# Autodesk Inventor assembly: CardGuideArray
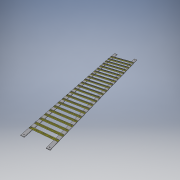
[picture p0: Inventor's stored thumbnail of the model, 180x180]
Saved by Autodesk Inventor 2018 (Build 220112000, 112)
## iProperties
Created: 2025-02-19
Part Number: CardGuideArray
Material: Všeobecné
Document SubType Name: Assembly
Designer: Jozko Mrkvicka
Author: Jozko Mrkvicka
## Documents named in this file (5)
- D:\05_Projekty\Projects_Inventor\Haluska9000\CardGuideArray-4-Inch.iam
- D:\05_Projekty\Projects_Inventor\Haluska9000\CardGuide.ipt
- D:\05_Projekty\Projects_Inventor\Haluska9000\Profile-Flat.ipt
- D:\05_Projekty\Projects_Inventor\Haluska9000\Profile-Flat\Profile-Flat#Cabinet-FerriteCore-Width.ipt
- D:\05_Projekty\Projects_Inventor\Haluska9000\CardGuide\CardGuide#4-inch.ipt
## Components (25 placed, 2 different names)
1. CardGuide#4-inch:1 — Proti sobě:3, Proti sobě:5, Proti sobě:91
2. Profile-Flat#Cabinet-FerriteCore-Width — Stejný směr:1, Stejný směr:2, Proti sobě:3, Proti sobě:5, Proti sobě:6, Proti sobě:7, Proti sobě:8, Proti sobě:9, Proti sobě:10, Proti sobě:11, Proti sobě:12, Proti sobě:13, Proti sobě:14, Proti sobě:15, Proti sobě:16, Proti sobě:17, Proti sobě:19, Proti sobě:20, Proti sobě:22, Proti sobě:23, Proti sobě:24, Proti sobě:25, Proti sobě:26, Proti sobě:27, Proti sobě:28, Proti sobě:29, Proti sobě:52, Proti sobě:53, Proti sobě:55, Proti sobě:56, Proti sobě:57, Proti sobě:58, Proti sobě:60, Proti sobě:73, Proti sobě:89, Proti sobě:94, Proti sobě:97, Proti sobě:101, Proti sobě:102
3. Profile-Flat#Cabinet-FerriteCore-Width:2 — Stejný směr:1, Stejný směr:2, Proti sobě:42, Proti sobě:43, Proti sobě:44, Proti sobě:45, Proti sobě:46, Proti sobě:47, Proti sobě:48, Proti sobě:50, Proti sobě:51, Proti sobě:72, Proti sobě:74, Proti sobě:77, Proti sobě:78, Proti sobě:79, Proti sobě:80, Proti sobě:81, Proti sobě:82, Proti sobě:83, Proti sobě:84, Proti sobě:85, Proti sobě:86, Proti sobě:87, Proti sobě:88, Proti sobě:90, Proti sobě:91, Proti sobě:92, Proti sobě:93, Proti sobě:95, Proti sobě:96, Proti sobě:98, Proti sobě:99, Proti sobě:100
4. CardGuide#4-inch:2 — Proti sobě:6, Proti sobě:19, Proti sobě:92
5. CardGuide#4-inch:3 — Proti sobě:7, Proti sobě:20, Proti sobě:87
6. CardGuide#4-inch:4 — Proti sobě:8, Proti sobě:29, Proti sobě:79
7. CardGuide#4-inch:5 — Proti sobě:9, Proti sobě:93, Proti sobě:94
8. CardGuide#4-inch:6 — Proti sobě:10, Proti sobě:88, Proti sobě:89
9. CardGuide#4-inch:7 — Proti sobě:11, Proti sobě:28, Proti sobě:80
10. CardGuide#4-inch:8 — Proti sobě:12, Proti sobě:27, Proti sobě:81
11. CardGuide#4-inch:9 — Proti sobě:13, Proti sobě:22, Proti sobě:86
12. CardGuide#4-inch:10 — Proti sobě:14, Proti sobě:26, Proti sobě:82
13. CardGuide#4-inch:11 — Proti sobě:15, Proti sobě:23, Proti sobě:83
14. CardGuide#4-inch:12 — Proti sobě:16, Proti sobě:25, Proti sobě:85
15. CardGuide#4-inch:13 — Proti sobě:17, Proti sobě:24, Proti sobě:84
16. CardGuide#4-inch:14 — Proti sobě:42, Proti sobě:52, Proti sobě:99
17. CardGuide#4-inch:15 — Proti sobě:44, Proti sobě:96, Proti sobě:97
18. CardGuide#4-inch:16 — Proti sobě:45, Proti sobě:55, Proti sobě:95
19. CardGuide#4-inch:17 — Proti sobě:43, Proti sobě:53, Proti sobě:98
20. CardGuide#4-inch:18 — Proti sobě:46, Proti sobě:56, Proti sobě:90
21. CardGuide#4-inch:19 — Proti sobě:48, Proti sobě:57, Proti sobě:78
22. CardGuide#4-inch:21 — Proti sobě:50, Proti sobě:60, Proti sobě:74
23. CardGuide#4-inch:22 — Proti sobě:47, Proti sobě:58, Proti sobě:77
24. CardGuide#4-inch:23 — Proti sobě:51, Proti sobě:72, Proti sobě:73
25. CardGuide#4-inch:24 — Proti sobě:100, Proti sobě:101, Proti sobě:102
## Relationships (71: Mate 69, Flush 2)
- Stejný směr:1 [Flush]: Profile-Flat#Cabinet-FerriteCore-Width ↔ Profile-Flat#Cabinet-FerriteCore-Width:2
- Stejný směr:2 [Flush]: Profile-Flat#Cabinet-FerriteCore-Width ↔ Profile-Flat#Cabinet-FerriteCore-Width:2
- Proti sobě:3 [Mate]: CardGuide#4-inch:1 ↔ Profile-Flat#Cabinet-FerriteCore-Width
- Proti sobě:5 [Mate]: CardGuide#4-inch:1 ↔ Profile-Flat#Cabinet-FerriteCore-Width
- Proti sobě:6 [Mate]: Profile-Flat#Cabinet-FerriteCore-Width ↔ CardGuide#4-inch:2
- Proti sobě:7 [Mate]: Profile-Flat#Cabinet-FerriteCore-Width ↔ CardGuide#4-inch:3
- Proti sobě:8 [Mate]: Profile-Flat#Cabinet-FerriteCore-Width ↔ CardGuide#4-inch:4
- Proti sobě:9 [Mate]: Profile-Flat#Cabinet-FerriteCore-Width ↔ CardGuide#4-inch:5
- Proti sobě:10 [Mate]: Profile-Flat#Cabinet-FerriteCore-Width ↔ CardGuide#4-inch:6
- Proti sobě:11 [Mate]: Profile-Flat#Cabinet-FerriteCore-Width ↔ CardGuide#4-inch:7
- Proti sobě:12 [Mate]: Profile-Flat#Cabinet-FerriteCore-Width ↔ CardGuide#4-inch:8
- Proti sobě:13 [Mate]: Profile-Flat#Cabinet-FerriteCore-Width ↔ CardGuide#4-inch:9
- Proti sobě:14 [Mate]: Profile-Flat#Cabinet-FerriteCore-Width ↔ CardGuide#4-inch:10
- Proti sobě:15 [Mate]: Profile-Flat#Cabinet-FerriteCore-Width ↔ CardGuide#4-inch:11
- Proti sobě:16 [Mate]: Profile-Flat#Cabinet-FerriteCore-Width ↔ CardGuide#4-inch:12
- Proti sobě:17 [Mate]: Profile-Flat#Cabinet-FerriteCore-Width ↔ CardGuide#4-inch:13
- Proti sobě:19 [Mate]: Profile-Flat#Cabinet-FerriteCore-Width ↔ CardGuide#4-inch:2
- Proti sobě:20 [Mate]: Profile-Flat#Cabinet-FerriteCore-Width ↔ CardGuide#4-inch:3
- Proti sobě:22 [Mate]: Profile-Flat#Cabinet-FerriteCore-Width ↔ CardGuide#4-inch:9
- Proti sobě:23 [Mate]: Profile-Flat#Cabinet-FerriteCore-Width ↔ CardGuide#4-inch:11
- Proti sobě:24 [Mate]: Profile-Flat#Cabinet-FerriteCore-Width ↔ CardGuide#4-inch:13
- Proti sobě:25 [Mate]: Profile-Flat#Cabinet-FerriteCore-Width ↔ CardGuide#4-inch:12
- Proti sobě:26 [Mate]: Profile-Flat#Cabinet-FerriteCore-Width ↔ CardGuide#4-inch:10
- Proti sobě:27 [Mate]: Profile-Flat#Cabinet-FerriteCore-Width ↔ CardGuide#4-inch:8
- Proti sobě:28 [Mate]: Profile-Flat#Cabinet-FerriteCore-Width ↔ CardGuide#4-inch:7
- Proti sobě:29 [Mate]: Profile-Flat#Cabinet-FerriteCore-Width ↔ CardGuide#4-inch:4
- Proti sobě:42 [Mate]: Profile-Flat#Cabinet-FerriteCore-Width:2 ↔ CardGuide#4-inch:14
- Proti sobě:43 [Mate]: Profile-Flat#Cabinet-FerriteCore-Width:2 ↔ CardGuide#4-inch:17
- Proti sobě:44 [Mate]: Profile-Flat#Cabinet-FerriteCore-Width:2 ↔ CardGuide#4-inch:15
- Proti sobě:45 [Mate]: Profile-Flat#Cabinet-FerriteCore-Width:2 ↔ CardGuide#4-inch:16
- Proti sobě:46 [Mate]: Profile-Flat#Cabinet-FerriteCore-Width:2 ↔ CardGuide#4-inch:18
- Proti sobě:47 [Mate]: Profile-Flat#Cabinet-FerriteCore-Width:2 ↔ CardGuide#4-inch:22
- Proti sobě:48 [Mate]: Profile-Flat#Cabinet-FerriteCore-Width:2 ↔ CardGuide#4-inch:19
- Proti sobě:50 [Mate]: Profile-Flat#Cabinet-FerriteCore-Width:2 ↔ CardGuide#4-inch:21
- Proti sobě:51 [Mate]: Profile-Flat#Cabinet-FerriteCore-Width:2 ↔ CardGuide#4-inch:23
- Proti sobě:52 [Mate]: Profile-Flat#Cabinet-FerriteCore-Width ↔ CardGuide#4-inch:14
- Proti sobě:53 [Mate]: Profile-Flat#Cabinet-FerriteCore-Width ↔ CardGuide#4-inch:17
- Proti sobě:55 [Mate]: Profile-Flat#Cabinet-FerriteCore-Width ↔ CardGuide#4-inch:16
- Proti sobě:56 [Mate]: Profile-Flat#Cabinet-FerriteCore-Width ↔ CardGuide#4-inch:18
- Proti sobě:57 [Mate]: Profile-Flat#Cabinet-FerriteCore-Width ↔ CardGuide#4-inch:19
- Proti sobě:58 [Mate]: Profile-Flat#Cabinet-FerriteCore-Width ↔ CardGuide#4-inch:22
- Proti sobě:60 [Mate]: Profile-Flat#Cabinet-FerriteCore-Width ↔ CardGuide#4-inch:21
- Proti sobě:72 [Mate]: Profile-Flat#Cabinet-FerriteCore-Width:2 ↔ CardGuide#4-inch:23
- Proti sobě:73 [Mate]: Profile-Flat#Cabinet-FerriteCore-Width ↔ CardGuide#4-inch:23
- Proti sobě:74 [Mate]: Profile-Flat#Cabinet-FerriteCore-Width:2 ↔ CardGuide#4-inch:21
- Proti sobě:77 [Mate]: Profile-Flat#Cabinet-FerriteCore-Width:2 ↔ CardGuide#4-inch:22
- Proti sobě:78 [Mate]: Profile-Flat#Cabinet-FerriteCore-Width:2 ↔ CardGuide#4-inch:19
- Proti sobě:79 [Mate]: Profile-Flat#Cabinet-FerriteCore-Width:2 ↔ CardGuide#4-inch:4
- Proti sobě:80 [Mate]: Profile-Flat#Cabinet-FerriteCore-Width:2 ↔ CardGuide#4-inch:7
- Proti sobě:81 [Mate]: Profile-Flat#Cabinet-FerriteCore-Width:2 ↔ CardGuide#4-inch:8
- Proti sobě:82 [Mate]: Profile-Flat#Cabinet-FerriteCore-Width:2 ↔ CardGuide#4-inch:10
- Proti sobě:83 [Mate]: Profile-Flat#Cabinet-FerriteCore-Width:2 ↔ CardGuide#4-inch:11
- Proti sobě:84 [Mate]: Profile-Flat#Cabinet-FerriteCore-Width:2 ↔ CardGuide#4-inch:13
- Proti sobě:85 [Mate]: Profile-Flat#Cabinet-FerriteCore-Width:2 ↔ CardGuide#4-inch:12
- Proti sobě:86 [Mate]: Profile-Flat#Cabinet-FerriteCore-Width:2 ↔ CardGuide#4-inch:9
- Proti sobě:87 [Mate]: Profile-Flat#Cabinet-FerriteCore-Width:2 ↔ CardGuide#4-inch:3
- Proti sobě:88 [Mate]: Profile-Flat#Cabinet-FerriteCore-Width:2 ↔ CardGuide#4-inch:6
- Proti sobě:89 [Mate]: Profile-Flat#Cabinet-FerriteCore-Width ↔ CardGuide#4-inch:6
- Proti sobě:90 [Mate]: Profile-Flat#Cabinet-FerriteCore-Width:2 ↔ CardGuide#4-inch:18
- Proti sobě:91 [Mate]: CardGuide#4-inch:1 ↔ Profile-Flat#Cabinet-FerriteCore-Width:2
- Proti sobě:92 [Mate]: Profile-Flat#Cabinet-FerriteCore-Width:2 ↔ CardGuide#4-inch:2
- Proti sobě:93 [Mate]: Profile-Flat#Cabinet-FerriteCore-Width:2 ↔ CardGuide#4-inch:5
- Proti sobě:94 [Mate]: Profile-Flat#Cabinet-FerriteCore-Width ↔ CardGuide#4-inch:5
- Proti sobě:95 [Mate]: Profile-Flat#Cabinet-FerriteCore-Width:2 ↔ CardGuide#4-inch:16
- Proti sobě:96 [Mate]: Profile-Flat#Cabinet-FerriteCore-Width:2 ↔ CardGuide#4-inch:15
- Proti sobě:97 [Mate]: Profile-Flat#Cabinet-FerriteCore-Width ↔ CardGuide#4-inch:15
- Proti sobě:98 [Mate]: Profile-Flat#Cabinet-FerriteCore-Width:2 ↔ CardGuide#4-inch:17
- Proti sobě:99 [Mate]: Profile-Flat#Cabinet-FerriteCore-Width:2 ↔ CardGuide#4-inch:14
- Proti sobě:100 [Mate]: Profile-Flat#Cabinet-FerriteCore-Width:2 ↔ CardGuide#4-inch:24
- Proti sobě:101 [Mate]: Profile-Flat#Cabinet-FerriteCore-Width ↔ CardGuide#4-inch:24
- Proti sobě:102 [Mate]: Profile-Flat#Cabinet-FerriteCore-Width ↔ CardGuide#4-inch:24
